# Autodesk Inventor assembly: angleBracket_MIR
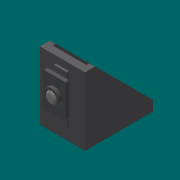
[picture p0: Inventor's stored thumbnail of the model, 180x180]
Saved by Autodesk Inventor 2016 SP1 (Build 200210100, 210)
## iProperties
Created: 2015-06-02
Part Number: angleBracket_MIR
Document SubType Name: Assembly
Designer: sawai
Author: Sawaiz Syed
## Documents named in this file (4)
- C:\Users\sawai\OneDrive\projects\modularRICH\testMount\frame\angleBracket_MIR.iam
- C:\Users\sawai\OneDrive\projects\modularRICH\testMount\frame\angleBracket_MIR.ipt
- C:\Users\sawai\OneDrive\projects\modularRICH\testMount\hardware\m5x10_MIR.ipt
- C:\Users\sawai\OneDrive\projects\modularRICH\testMount\hardware\m5TNut_MIR.ipt
## Components (5 placed, 3 different names)
1. angleBracket_MIR:1 — Mate:14, Mate:12, Mate:15, Mate:13, Angle:2, Mate:9, Angle:3, Mate:11
2. m5x10_MIR:1 — Mate:14, Mate:12, Mate:16
3. m5x10_MIR:2 — Mate:15, Mate:13, Mate:17
4. m5TNut_MIR:1 — Mate:16, Angle:2, Mate:9
5. m5TNut_MIR:2 — Mate:17, Angle:3, Mate:11
## Relationships (10: Mate 8, Angle 2)
- Mate:14: angleBracket_MIR:1 ↔ m5x10_MIR:1
- Mate:12: angleBracket_MIR:1 ↔ m5x10_MIR:1
- Mate:15: angleBracket_MIR:1 ↔ m5x10_MIR:2
- Mate:13: angleBracket_MIR:1 ↔ m5x10_MIR:2
- Mate:16: m5x10_MIR:1 ↔ m5TNut_MIR:1
- Angle:2 (0 deg): angleBracket_MIR:1 ↔ m5TNut_MIR:1
- Mate:9 (2 mm): angleBracket_MIR:1 ↔ m5TNut_MIR:1
- Mate:17: m5x10_MIR:2 ↔ m5TNut_MIR:2
- Angle:3 (0 deg): angleBracket_MIR:1 ↔ m5TNut_MIR:2
- Mate:11 (2 mm): angleBracket_MIR:1 ↔ m5TNut_MIR:2
